# Autodesk Inventor assembly: Assembly
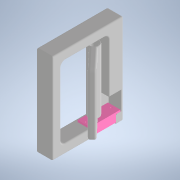
[picture p0: Inventor's stored thumbnail of the model, 180x180]
Saved by Autodesk Inventor 2020.1 (Build 241239000, 239)
## iProperties
Created: 2022-04-03
Part Number: Assembly
Document SubType Name: Assembly
Designer: OEM
Author: OEM
## Documents named in this file (4)
- C:\Users\OEM\Desktop\HandSomething\Drzwi_CAD\Assembly.iam
- C:\Users\OEM\Desktop\HandSomething\Drzwi_CAD\Framuga.ipt
- C:\Users\OEM\Desktop\HandSomething\Drzwi_CAD\servo_sub.ipt
- C:\Users\OEM\Desktop\HandSomething\Drzwi_CAD\Drzwi.ipt
## Components (3 placed, 3 different names)
1. Framuga:2 — Mate:1, Mate:2, Mate:3
2. servo_sub:2 — Mate:1, Mate:2, Mate:3, Mate:4, Mate:5
3. Drzwi:1 — Mate:4, Mate:5
## Relationships (5: Mate 5)
- Mate:1: Framuga:2 ↔ servo_sub:2
- Mate:2: Framuga:2 ↔ servo_sub:2
- Mate:3: Framuga:2 ↔ servo_sub:2
- Mate:4: servo_sub:2 ↔ Drzwi:1
- Mate:5: servo_sub:2 ↔ Drzwi:1
